# Autodesk Inventor assembly: Dresser Frame
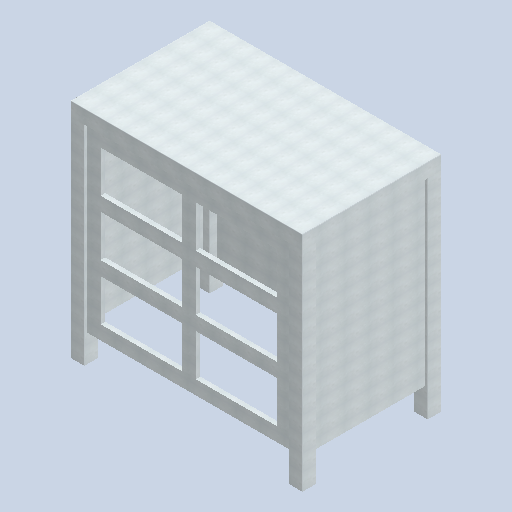
[picture p0: Inventor's stored thumbnail of the model, 512x512]
Saved by Autodesk Inventor 2022 (Build 260153000, 153)
## iProperties
Company: Jay's Dressers
RuleStatus: InUse
Created: 2021-10-04
Document SubType Name: Assembly
Designer: Admin
Author: Admin
Title: Dresser Frame
## Documents named in this file (7)
- C:\Users\Admin\source\repos\DresserWebApplication\DresserAutomationPlugin\Resources\Dresser Base Model\Dresser Frame.iam
- C:\Users\Admin\source\repos\DresserWebApplication\DresserAutomationPlugin\Resources\Dresser Base Model\Leg.ipt
- C:\Users\Admin\source\repos\DresserWebApplication\DresserAutomationPlugin\Resources\Dresser Base Model\Top Panel.ipt
- C:\Users\Admin\source\repos\DresserWebApplication\DresserAutomationPlugin\Resources\Dresser Base Model\Dresser SKELETON.ipt
- C:\Users\Admin\source\repos\DresserWebApplication\DresserAutomationPlugin\Resources\Dresser Base Model\Front Panel.ipt
- C:\Users\Admin\source\repos\DresserWebApplication\DresserAutomationPlugin\Resources\Dresser Base Model\Back Panel.ipt
- C:\Users\Admin\source\repos\DresserWebApplication\DresserAutomationPlugin\Resources\Dresser Base Model\Side Panel.ipt
## Components (10 placed, 6 different names)
1. Dresser SKELETON:1 — Mate:5, Flush:7, Flush:8, Mate:8, Mate:9, Mate:10, Flush:5, Flush:6
2. Leg:1
3. Leg:2 — Flush:1, Flush:8, Mate:8
4. Leg:3 — Flush:2, Mate:9, Mate:10
5. Leg:4 — Flush:3, Mate:5, Flush:7
6. Top Panel:1
7. Front Panel:1
8. Back Panel:1
9. Side Panel:1 — Flush:4
10. Side Panel:2 — Flush:4, Flush:5, Flush:6
## Relationships (12: Flush 8, Mate 4)
- Flush:1: Leg:2
- Flush:2: Leg:3
- Flush:3: Leg:4
- Mate:5: Dresser SKELETON:1 ↔ Leg:4
- Flush:7: Dresser SKELETON:1 ↔ Leg:4
- Flush:8: Dresser SKELETON:1 ↔ Leg:2
- Mate:8: Dresser SKELETON:1 ↔ Leg:2
- Mate:9: Dresser SKELETON:1 ↔ Leg:3
- Mate:10: Dresser SKELETON:1 ↔ Leg:3
- Flush:4: Side Panel:1 ↔ Side Panel:2
- Flush:5: Dresser SKELETON:1 ↔ Side Panel:2
- Flush:6: Dresser SKELETON:1 ↔ Side Panel:2
